# Autodesk Inventor assembly: GlidelejrehusAssembly
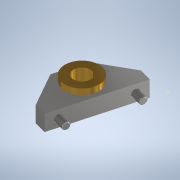
[picture p0: Inventor's stored thumbnail of the model, 180x180]
Saved by Autodesk Inventor 2022.2 (Build 262287010, 287A)
## iProperties
Created: 2022-04-19
Part Number: GlidelejrehusAssembly
Document SubType Name: Assembly
Designer: Finn Oriwohl
Author: Finn Oriwohl
## Documents named in this file (3)
- C:\Users\Finn Oriwohl\Documents\htx\1g g\BeerCart-CAD-Inventor\Workspaces\Workspace\beercart assembly - mekatronik\Frame\GlidelejrehusAssembly.iam
- C:\Users\Finn Oriwohl\Documents\htx\1g g\BeerCart-CAD-Inventor\Workspaces\Workspace\Build drawings\Glidelejrehus.ipt
- C:\Users\Finn Oriwohl\Documents\htx\1g g\BeerCart-CAD-Inventor\Workspaces\Workspace\Build drawings\glide lejre bushing.ipt
## Components (2 placed, 2 different names)
1. Glidelejrehus:1
2. glide lejre bushing:1
## Relationships (2: Flush 1, Insert 1)
- [Flush]: Glidelejrehus:1 ↔ glide lejre bushing:1
- [Insert]: Glidelejrehus:1 ↔ glide lejre bushing:1
